# Autodesk Inventor assembly: Baugruppe1
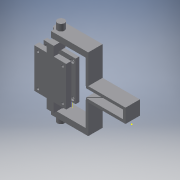
[picture p0: Inventor's stored thumbnail of the model, 180x180]
Saved by Autodesk Inventor 2018.3 (Build 223284000, 284)
## iProperties
Created: 2018-11-22
Part Number: Baugruppe1
Material: Generisch
Document SubType Name: Assembly
Designer: pgmadmin
Author: pgmadmin
## Documents named in this file (5)
- H:\Homeverzeichnis\CAD\FReiburg Seminar- in bearbeitung\Strahlenteiler 25.10\Baugruppe1.iam
- H:\Homeverzeichnis\CAD\FReiburg Seminar- in bearbeitung\Strahlenteiler 25.10\Neue Grundplatte.ipt
- H:\Homeverzeichnis\CAD\FReiburg Seminar- in bearbeitung\Strahlenteiler 25.10\Spieghalter 2.0.ipt
- H:\Homeverzeichnis\CAD\FReiburg Seminar- in bearbeitung\Strahlenteiler 25.10\Klemme.ipt
- H:\Homeverzeichnis\CAD\FReiburg Seminar- in bearbeitung\Strahlenteiler 25.10\Spiegelhalter_klein.ipt
## Components (5 placed, 4 different names)
1. Neue Grundplatte:1 — Passend:1, Passend:3, Passend:5
2. Spieghalter 2.0:1 — Passend:1, Passend:2, Passend:4, Starr:1
3. Klemme:1 — Passend:2, Passend:3
4. Klemme:2 — Passend:4, Passend:5
5. Spiegelhalter_klein:1 — Starr:1
## Relationships (6: Mate 5, WeldJoint 1)
- Passend:1 [Mate]: Neue Grundplatte:1 ↔ Spieghalter 2.0:1
- Passend:2 [Mate]: Spieghalter 2.0:1 ↔ Klemme:1
- Passend:3 [Mate]: Neue Grundplatte:1 ↔ Klemme:1
- Passend:4 [Mate]: Spieghalter 2.0:1 ↔ Klemme:2
- Passend:5 [Mate]: Neue Grundplatte:1 ↔ Klemme:2
- Starr:1 [WeldJoint] (6 mm): Spieghalter 2.0:1 ↔ Spiegelhalter_klein:1
